# Autodesk Inventor assembly: Form
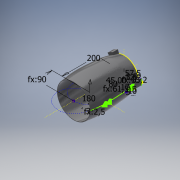
[picture p0: Inventor's stored thumbnail of the model, 180x180]
Saved by Autodesk Inventor 2019.1 (Build 231200000, 200)
## iProperties
Created: 2018-07-24
Part Number: Form
Material: Generisch
Document SubType Name: Assembly
Designer: JochenAlt
Author: JochenAlt
## Documents named in this file (3)
- D:\Projects\Ondine\CAD\Form.iam
- D:\Projects\Ondine\CAD\Form.ipt
- D:\Projects\Ondine\CAD\Spindle\SpindleThreadLong.ipt
## Components (4 placed, 2 different names)
1. Form:1 — Passend:1, Passend:2, Passend:3, Passend:4, Passend:5, Passend:6, Winkel:1, Winkel:2, Winkel:3
2. SpindleThread:1 — Passend:1, Passend:2, Winkel:2
3. SpindleThread:2 — Passend:3, Passend:4, Winkel:3
4. SpindleThread:3 — Passend:5, Passend:6, Winkel:1
## Relationships (9: Mate 6, Angle 3)
- Passend:1 [Mate]: Form:1 ↔ SpindleThread:1
- Passend:2 [Mate]: Form:1 ↔ SpindleThread:1
- Passend:3 [Mate]: Form:1 ↔ SpindleThread:2
- Passend:4 [Mate]: Form:1 ↔ SpindleThread:2
- Passend:5 [Mate]: Form:1 ↔ SpindleThread:3
- Passend:6 [Mate]: Form:1 ↔ SpindleThread:3
- Winkel:1 [Angle] (0 deg): Form:1 ↔ SpindleThread:3
- Winkel:2 [Angle] (0 deg): Form:1 ↔ SpindleThread:1
- Winkel:3 [Angle] (0 deg): Form:1 ↔ SpindleThread:2
